# Autodesk Inventor assembly: ensamble 3
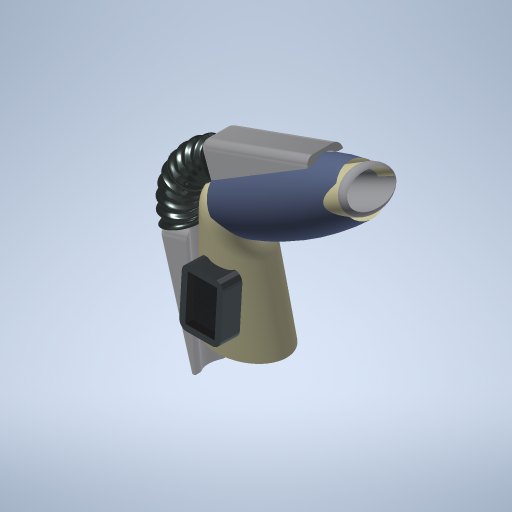
[picture p0: Inventor's stored thumbnail of the model, 512x512]
Saved by Autodesk Inventor 2023 (Build 270158000, 158)
## iProperties
Created: 2022-10-07
Part Number: ensamble 3
Document SubType Name: Assembly
Designer: Xiaba
Author: Xiaba
## Documents named in this file (5)
- C:\Users\Xiaba\Desktop\Funbio\INVENTOR\ensamble 3.iam
- C:\Users\Xiaba\Desktop\Funbio\INVENTOR\partes de plastico.ipt
- C:\Users\Xiaba\Desktop\Funbio\INVENTOR\pat 1 brazo.ipt
- C:\Users\Xiaba\Desktop\Funbio\INVENTOR\resorte.ipt
- C:\Users\Xiaba\Desktop\Funbio\INVENTOR\bateria pat 1.ipt
## Components (6 placed, 4 different names)
1. partes de plastico:1 — Mate:1
2. partes de plastico:2 — Mate:2
3. pat 1 brazo:1
4. resorte:1 — Mate:1
5. resorte:2 — Mate:2
6. bateria pat 1:1
## Relationships (2: Mate 2)
- Mate:1: partes de plastico:1 ↔ resorte:1
- Mate:2: partes de plastico:2 ↔ resorte:2
